# Autodesk Inventor assembly: cover_final_assembly
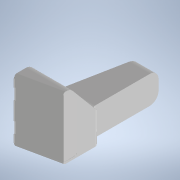
[picture p0: Inventor's stored thumbnail of the model, 180x180]
Saved by Autodesk Inventor 2021 (Build 250183000, 183)
## iProperties
Created: 2021-06-25
Part Number: cover_final_assembly
Document SubType Name: Assembly
## Documents named in this file (4)
- C:\Users\ocon0143\OneDrive - Flinders\Advn Mech Design Shared\6_Development\2_Design\inventor\cover\cover_final_assembly.iam
- C:\Users\ocon0143\OneDrive - Flinders\Advn Mech Design Shared\6_Development\2_Design\inventor\vehicle_wheelchair\wheelchair\wheelchair_box_extended.ipt
- C:\Users\ocon0143\OneDrive - Flinders\Advn Mech Design Shared\6_Development\2_Design\inventor\cover\cover_open_door.ipt
- C:\Users\ocon0143\OneDrive - Flinders\Advn Mech Design Shared\6_Development\2_Design\inventor\cover\linear_actuator_as.iam
## Components (3 placed, 3 different names)
1. wheelchair_box_extended:1 — Mate:1, Flush:1, Flush:2, Mate:2, Flush:3, Mate:3, Mate:4
2. cover_open_door:1 — Mate:2, Flush:3, Mate:5
3. linear_actuator_as:1 [sub-assembly] — Mate:3, Mate:4, Mate:5
## Relationships (8: Mate 5, Flush 3)
- Mate:1: wheelchair_box_extended:1
- Flush:1: wheelchair_box_extended:1
- Flush:2: wheelchair_box_extended:1
- Mate:2: wheelchair_box_extended:1 ↔ cover_open_door:1
- Flush:3 (50 mm): wheelchair_box_extended:1 ↔ cover_open_door:1
- Mate:3: wheelchair_box_extended:1 ↔ linear_actuator_as:1
- Mate:4 (60 mm): wheelchair_box_extended:1 ↔ linear_actuator_as:1
- Mate:5: cover_open_door:1 ↔ linear_actuator_as:1
